# Autodesk Inventor assembly: hegnspæl, oppe, top
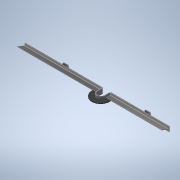
[picture p0: Inventor's stored thumbnail of the model, 180x180]
Saved by Autodesk Inventor 2020.1 (Build 241239000, 239)
## iProperties
Created: 2019-09-30
Part Number: hegnspæl, oppe, top
Document SubType Name: Assembly
Designer: Kristoffer Ek
Mass: 1821.47 g
Surface Area: 1100.09 cm^2
Volume: 232.034 cm^3
Density: 7.85 g/cm^3
_SolveAssemblyDoc: Frame Generator Solve Assembly
_Version: 15.0.0
Author: gust3763
## Documents named in this file (10)
- Y:\trappe\hegn\hegnspæl, oppe, top.iam
- hegnspæl.iam
- Y:\trappe\hegn\t-profil.ipt
- Y:\trappe\hegn\t-profil\Frame\Frame0002.iam
- Y:\trappe\hegn\hage.ipt
- Y:\trappe\hegn\bue.ipt
- Y:\trappe\hegn\bukket del.ipt
- Y:\trappe\hegn\gevindmuffe.ipt
- C:\Users\stoffer\Documents\Inventor\Content Center Files\R2020\en-US\ISO 4762(2)\ISO 4762 - M6 x 16ISO.ipt
- Y:\trappe\trappe.xlsx
## Components (8 placed, 7 different names)
1. t-profil:1 — Flush:9
2. Frame0002:1 [sub-assembly] — Mate:1, Mate:3, Angle:1, Mate:4, Angle:2, Flush:5, Mate:5, Mate:9, Flush:10, Flush:11, Mate:11, Mate:12, Flush:12, Mate:13, Mate:14, Mate:16
3. hage:1 — Mate:1, Mate:5, Flush:7, Flush:8, Mate:10, Flush:13
4. hage:4 — Flush:7, Mate:9, Mate:10, Flush:13
5. bue:1 — Flush:10, Flush:11
6. bukket del:1 — Mate:11, Mate:12, Flush:12
7. gevindmuffe:1 — Mate:13, Mate:14, Mate:15
8. ISO 4762 M6 x 16:1 — Mate:15, Mate:16
## Relationships (22: Mate 12, Flush 8, Angle 2)
- Mate:1: Frame0002:1 ↔ hage:1
- Mate:3: Frame0002:1
- Angle:1 (0 deg): Frame0002:1
- Mate:4: Frame0002:1
- Angle:2 (0 deg): Frame0002:1
- Flush:5: Frame0002:1
- Mate:5 (135 mm): Frame0002:1 ↔ hage:1
- Flush:7: hage:1 ↔ hage:4
- Mate:9: Frame0002:1 ↔ hage:4
- Flush:8 (385 mm): hage:1
- Mate:10 (500 mm): hage:1 ↔ hage:4
- Flush:9: t-profil:1
- Flush:10: Frame0002:1 ↔ bue:1
- Flush:11: Frame0002:1 ↔ bue:1
- Mate:11: Frame0002:1 ↔ bukket del:1
- Mate:12 (4 mm): Frame0002:1 ↔ bukket del:1
- Flush:12: Frame0002:1 ↔ bukket del:1
- Flush:13: hage:1 ↔ hage:4
- Mate:13: Frame0002:1 ↔ gevindmuffe:1
- Mate:14: Frame0002:1 ↔ gevindmuffe:1
- Mate:15: gevindmuffe:1 ↔ ISO 4762 M6 x 16:1
- Mate:16: Frame0002:1 ↔ ISO 4762 M6 x 16:1
## Named parameters: trappevinkel = 34.3 deg, trappestifter_dia = 25 mm, trappestifter_huldia = 25.8 mm, trappestifter_skraa_huldia = 26.6 mm, trappestifter_laengde = 228 mm, perforeringsbredde = 6 mm, perforeringshulprocent = 80 mm, perforeringshullaengde = 62.8 mm, perforeringshullaengde_top = 61 mm, perforeringshullaengde_bund = 61.6 mm, perforeringsoffset = 8 mm, perforeringsoffset_top = 8 mm, perforeringsoffset_bund = 8 mm, laskehul_dia = 13 mm, haandfang_offset_fra_top = 90 mm, balusterhul_udvidelse = 1 mm, pladetykkelse = 3 mm, trinhoejde = 100 mm, trinbredde = 1884 mm
